# Autodesk Inventor assembly: Shooter Assembly v2
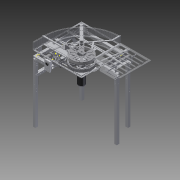
[picture p0: Inventor's stored thumbnail of the model, 180x180]
Saved by Autodesk Inventor 2013 (Build 170138000, 138)
## iProperties
Created: 2013-01-15
Part Number: Shooter Assembly v2
Document SubType Name: Assembly
Designer: actoennies
Mass: 9919.81 g
Surface Area: 30757 cm^2
Volume: 4898.75 cm^3
Density: 2.02497 g/cm^3
Author: actoennies
## Documents named in this file (53)
- C:\Users\Arpan\Documents\GitHub\frc2013CAD\Launcher\Shooter\Shooter Assembly v2.iam
- C:\Users\Arpan\Documents\GitHub\frc2013CAD\Launcher\Shooter\Bearing Mount v1.ipt
- C:\Users\Arpan\Documents\GitHub\frc2013CAD\Launcher\Shooter\Outer Rail v1.ipt
- C:\Users\Arpan\Documents\GitHub\frc2013CAD\Launcher\Shooter\Runner Rails v2.ipt
- C:\Users\Arpan\Documents\GitHub\frc2013CAD\Launcher\Shooter\Bearing.ipt
- C:\Users\Arpan\Documents\GitHub\frc2013CAD\Launcher\Shooter\Flywheel Assembly.iam
- C:\Users\Arpan\Documents\GitHub\frc2013CAD\Launcher\Shooter\Shooter Mounter.ipt
- C:\Users\Arpan\Documents\GitHub\frc2013CAD\Launcher\Shooter\Bearing Mount 2 v1.ipt
- C:\Users\Arpan\Documents\GitHub\frc2013CAD\Launcher\Shooter\Shorter Shaft.ipt
- C:\Users\Arpan\Documents\GitHub\frc2013CAD\Launcher\Shooter\Spacer Rube.ipt
- C:\Users\Arpan\Documents\GitHub\frc2013CAD\Launcher\Shooter\Edge Mount.ipt
- C:\Users\Arpan\Documents\GitHub\frc2013CAD\Launcher\Shooter\Square Tube.ipt
- C:\Users\Arpan\Documents\GitHub\frc2013CAD\Launcher\Shooter\Flange Bearing Mount Tower.ipt
- C:\Users\Arpan\Documents\GitHub\frc2013CAD\Launcher\Shooter\Flange Bearing Mount Tower Mirror.ipt
- C:\Users\Arpan\Documents\GitHub\frc2013CAD\Launcher\Shooter\Bearing Mount Top.ipt
- C:\Users\Arpan\Documents\GitHub\frc2013CAD\Launcher\Shooter\Square Motor Mount.ipt
- C:\Users\Arpan\Documents\GitHub\frc2013CAD\Launcher\Shooter\Shooter Assembly v2\Design Accelerator\Spur Gears1.iam
- C:\Users\Arpan\Documents\GitHub\frc2013CAD\Launcher\Parts\Imported Components\Snow Blower Motor\Snow Blower Motor.iam
- C:\Users\Arpan\Documents\GitHub\frc2013CAD\Launcher\Shooter\Snowblower Motor Mount.ipt
- C:\Users\Arpan\Documents\GitHub\frc2013CAD\Launcher\Shooter\8mm shaft.ipt
- C:\Users\Arpan\Documents\GitHub\frc2013CAD\Launcher\Shooter\CIM Bearing.ipt
- C:\Users\Arpan\Documents\GitHub\frc2013CAD\Launcher\Parts\8 Plaction Wheel.iam
- C:\Users\Arpan\Documents\GitHub\frc2013CAD\Launcher\Shooter\Square Tube 2.ipt
- C:\Users\Arpan\Documents\GitHub\frc2013CAD\Launcher\Parts\CIM Motor\Motors_FR801-001.iam
- C:\Users\Arpan\Documents\GitHub\frc2013CAD\Launcher\Shooter\Cim Mount.ipt
- C:\Users\Arpan\Documents\GitHub\frc2013CAD\Launcher\Shooter\Hub v1.ipt
- C:\Users\Arpan\Documents\GitHub\frc2013CAD\Launcher\Shooter\Camera Traffic Light Mount.ipt
- C:\Users\Arpan\Documents\GitHub\frc2013CAD\Launcher\Shooter\Square Tube 3.ipt
- C:\Users\Arpan\Documents\GitHub\frc2013CAD\Launcher\Shooter\edge mount shortened.ipt
- C:\Users\Arpan\Documents\GitHub\frc2013CAD\Launcher\Shooter\Camera.ipt
- C:\Users\Arpan\Documents\GitHub\frc2013CAD\Launcher\Shooter\Square Tube 6.ipt
- C:\Users\Arpan\Documents\GitHub\frc2013CAD\Launcher\Parts\NR-025_5-D(F,D-770).iam
- C:\Users\Arpan\Documents\GitHub\frc2013CAD\Launcher\Shooter\Upper Rails.ipt
- C:\Users\Arpan\Documents\GitHub\frc2013CAD\Launcher\Hopper New\Hopper Assembly.iam
- C:\Users\Arpan\Documents\GitHub\frc2013CAD\Launcher\Hopper New\Puller Mechanism.ipt
- C:\Users\Arpan\Documents\GitHub\frc2013CAD\Launcher\Shooter\Cylinder Mount 2.ipt
- C:\Users\Arpan\Documents\GitHub\frc2013CAD\Launcher\Shooter\Cylinder Mount.ipt
- C:\Users\Arpan\Documents\GitHub\frc2013CAD\Launcher\Parts\Imported Components\E3-X-315-X-D-3-X\E3-X-315-X-D-3-X.ipt
- C:\Users\Arpan\Documents\GitHub\frc2013CAD\Launcher\Shooter\Encoder Mounting.ipt
- C:\Users\Arpan\Documents\GitHub\frc2013CAD\Launcher\Hopper New\Backboard.ipt
- C:\Users\Arpan\Documents\GitHub\frc2013CAD\Launcher\Hopper New\Mount.ipt
- C:\Users\Arpan\Documents\GitHub\frc2013CAD\Launcher\Shooter\Gusset.ipt
- C:\Users\Arpan\Documents\GitHub\frc2013CAD\Launcher\Shooter\Gusset 2.ipt
- C:\Users\Arpan\Documents\GitHub\frc2013CAD\Launcher\Shooter\Gusset 3.ipt
- C:\Users\Arpan\Documents\GitHub\frc2013CAD\Launcher\Shooter\Gusset 4.ipt
- C:\Users\Arpan\Documents\GitHub\frc2013CAD\Launcher\Shooter\Inner Mount.ipt
- C:\Users\Arpan\Documents\GitHub\frc2013CAD\Launcher\Shooter\Gusset 5.ipt
- C:\Users\Arpan\Documents\GitHub\frc2013CAD\Launcher\Shooter\Hard Stop.ipt
- C:\Users\Arpan\Documents\GitHub\frc2013CAD\Launcher\Shooter\Gusset Connector 2.ipt
- C:\Users\Arpan\Documents\GitHub\frc2013CAD\Launcher\Shooter\Pneumatic Puller Mount.ipt
- C:\Users\Arpan\Documents\GitHub\frc2013CAD\Launcher\Shooter\L-Channel Strenght.ipt
- C:\Users\Arpan\Documents\GitHub\frc2013CAD\Launcher\Shooter\Gear for Angle.ipt
- C:\Users\Arpan\Documents\GitHub\frc2013CAD\Launcher\Shooter\Encoder Mount 2.ipt
## Components (78 placed, 52 different names)
1. Bearing Mount v1:1 — Insert:13, Insert:26, Insert:27, Mate:62, Mate:63, Flush:70, Insert:60, Insert:61, Mate:167
2. Outer Rail v1:1 — Insert:13, Insert:47, Insert:48, Flush:70, Mate:165
3. Runner Rails v2:1 — Insert:60, Insert:61, Mate:166, Angle:11, Flush:75, Mate:180, Mate:181, Flush:77
4. Flywheel Assembly:1 [sub-assembly] — Mate:61, Flush:30, Mate:68, Flush:31
5. Shooter Mounter:1 — Insert:26, Insert:27, Insert:34, Flush:11, Insert:35, Insert:36, Insert:37, Insert:38, Flush:19, Mate:45, Flush:40, Flush:64, Flush:72, Angle:6, Mate:176, Flush:76, Mate:183, Flush:78, Mate:226, Flush:114, Flush:115, Mate:229, Mate:230, Flush:116, Mate:232, Flush:117, Mate:236, Flush:118, Flush:119, Mate:238, Insert:75
6. Spacer Rube:1 — Insert:34, Flush:11
7. Bearing Mount 2 v1:1 — Insert:37, Insert:38, Insert:40
8. Bearing Mount 2 v1:2 — Insert:35, Insert:36, Insert:39
9. Bearing:3 — Insert:40, Flush:13, Mate:14, Mate:15
10. Bearing:4 — Insert:39, Flush:12, Mate:12, Mate:13, Mate:36, Mate:44
11. Shorter Shaft:1 — Flush:12, Mate:12, Mate:13, Mate:37
12. Shorter Shaft:2 — Flush:13, Mate:14, Mate:15, Mate:38
13. Edge Mount:2 — Flush:34, Mate:104, Flush:48, Mate:106, Flush:68, Mate:174, Flush:74, Mate:220, Mate:222
14. Square Tube:2 — Flush:19, Flush:23, Mate:52, Flush:27, Mate:81, Flush:32, Mate:93, Flush:41, Flush:42, Mate:125, Mate:126, Mate:130, Flush:50, Mate:169, Mate:192, Flush:83, Mate:203, Flush:88, Mate:214, Mate:217, Flush:103, Flush:112, Insert:71, Insert:72
15. Flange Bearing Mount Tower:1 — Insert:43, Flush:112, Flush:113
16. Bearing:5 — Insert:43, Mate:36, Mate:37
17. Flange Bearing Mount Tower Mirror:1 — Flush:55, Mate:135, Flush:111, Insert:70
18. Bearing:6 — Mate:38, Insert:70
19. Bearing Mount Top:1 — Insert:47, Insert:48, Mate:65, Mate:66, Mate:68, Mate:162, Mate:163, Mate:164
20. Square Motor Mount:1 — Flush:23, Mate:47, Mate:51, Flush:27, Mate:131, Mate:197, Mate:198, Flush:86, Flush:96, Flush:106
21. Spur Gears:1 [sub-assembly] — Mate:44, Mate:45, Flush:25, Mate:46, Angle:2, Flush:64, Angle:6, Angle:10, Mate:227, Mate:228, Mate:231, Mate:233, Flush:120, Mate:239
22. Snow Blower Motor:1 [sub-assembly] — Flush:25, Mate:46, Angle:2, Insert:50, Insert:51
23. Snowblower Motor Mount:1 — Insert:50, Insert:51, Mate:47, Mate:51, Mate:52, Mate:240, Insert:76, Insert:78, Insert:79
24. 8mm shaft:1 — Mate:61, Flush:30, Mate:67, Flush:31, Mate:82, Mate:83, Mate:84, Mate:86, Mate:167, Insert:64
25. CIM Bearing:1 — Mate:65, Mate:66, Mate:67
26. CIM Bearing:2 — Mate:62, Mate:63, Insert:56
27. 8 Plaction Wheel:1 [sub-assembly] — Mate:88, Mate:89, Mate:90, Mate:91, Mate:92
28. Square Tube 2:1 — Mate:81, Flush:32, Flush:34, Mate:106, Mate:124, Flush:49, Mate:126, Mate:173, Mate:186, Flush:80, Mate:193, Mate:216, Mate:219, Flush:104, Flush:111, Flush:113
29. Motors_FR801-001:1 [sub-assembly] — Mate:82, Mate:83, Mate:84, Mate:143, Mate:144, Mate:145
30. Cim Mount:1 — Flush:40, Mate:143, Mate:144, Mate:145
31. Hub v1:1 — Mate:88, Mate:89, Mate:90, Flush:38
32. Hub v1:2 — Mate:91, Flush:38, Mate:92, Insert:56
33. Camera Traffic Light Mount:1 — Mate:93, Flush:41, Flush:42, Mate:127, Mate:128, Mate:129, Mate:202, Mate:211, Angle:15
34. Square Tube 3:1 — Mate:104, Flush:48, Flush:55, Mate:135, Mate:173, Mate:174, Flush:74, Mate:175, Mate:187, Mate:206, Flush:90, Mate:221, Flush:105, Flush:110
35. edge mount shortened:1 — Mate:124, Mate:125, Flush:49, Mate:196, Flush:85, Mate:215, Flush:102, Mate:218, Mate:223, Flush:107
36. Camera:1 — Mate:127, Mate:128, Mate:129
37. Edge Mount:3 — Mate:130, Mate:131, Flush:50, Mate:199, Mate:209, Flush:97, Mate:212, Flush:100, Mate:213, Flush:101
38. Square Tube 6:1 — Mate:175, Flush:91, Mate:207, Flush:93, Mate:208, Flush:94, Flush:95, Flush:110, Mate:224, Insert:73, Insert:74
39. Upper Rails:1 — Mate:162, Mate:163, Mate:164
40. Hopper Assembly:1 [sub-assembly] — Flush:72, Mate:165, Mate:166, Flush:75, Angle:12, Mate:178, Mate:179
41. Puller Mechanism:1 — Insert:69, Angle:12, Mate:237
42. Cylinder Mount 2:1 — Angle:10, Mate:169, Angle:13, Mate:182, Mate:183, Flush:78
43. Cylinder Mount:1 — Mate:176, Flush:76, Mate:177, Insert:66, Insert:67
44. E3-X-315-X-D-3-X:1 — Insert:64, Insert:65
45. Encoder Mounting:1 — Insert:65, Angle:11
46. NR-025_5-D(F,D-770):1 [sub-assembly] — Mate:177, Insert:66, Insert:67, Insert:69, Angle:13, Mate:182
47. Backboard:1 — Mate:178, Mate:179
48. Mount:1 — Mate:180, Mate:181, Flush:77
49. Gusset:3 — Mate:186, Flush:80, Mate:187
50. Gusset:4 — Mate:196, Mate:197, Flush:85
51. Gusset:5 — Mate:192, Mate:193, Flush:83
52. Gusset:8 — Mate:198, Mate:199, Flush:86
53. Gusset:10 — Mate:202, Mate:203, Flush:88
54. Gusset 2:1 — Mate:206, Flush:90, Flush:91
55. Gusset 3:2 — Mate:209, Flush:96, Flush:97
56. Gusset 3:3 — Mate:208, Flush:94, Flush:95, Flush:108
57. Gusset 3:4 — Mate:207, Flush:93, Mate:225
58. Gusset 4:1 — Mate:211, Mate:212, Flush:100
59. Gusset 4:2 — Mate:213, Flush:101, Mate:214
60. Gusset 4:3 — Mate:217, Mate:218, Flush:103
61. Gusset 4:4 — Mate:215, Flush:102, Mate:216
62. Gusset 4:5 — Mate:219, Mate:220, Flush:104
63. Gusset 4:6 — Mate:221, Mate:222, Flush:105
64. Gusset 3:5 — Mate:223, Flush:106, Flush:107
65. Inner Mount:1 — Flush:108, Mate:224, Mate:225
66. Gusset 5:1 — Flush:115, Mate:228, Mate:229
67. Gusset 5:2 — Mate:226, Mate:227, Flush:114
68. Gusset 5:3 — Mate:230, Mate:231, Flush:116
69. Gusset 5:4 — Mate:232, Mate:233, Flush:117
70. Hard Stop:1 — Insert:71, Insert:72
71. Gusset Connector 2:1 — Insert:73, Insert:74
72. Pneumatic Puller Mount:1 — Mate:236, Flush:118, Mate:237
73. L-Channel Strenght:1 — Flush:119, Mate:238, Insert:75, Angle:15
74. Gear for Angle:1 — Flush:120, Mate:239, Mate:240, Flush:121
75. CIM Bearing:3 — Insert:76, Insert:77
76. 8mm shaft:2 — Insert:77, Flush:121
77. E3-X-315-X-D-3-X:2 — Insert:80, Angle:14
78. Encoder Mount 2:1 — Insert:78, Insert:79, Insert:80, Angle:14
## Relationships (208: Mate 105, Flush 61, Insert 34, Angle 8)
- Insert:13: Bearing Mount v1:1 ↔ Outer Rail v1:1
- Insert:26: Bearing Mount v1:1 ↔ Shooter Mounter:1
- Insert:27: Bearing Mount v1:1 ↔ Shooter Mounter:1
- Insert:34: Shooter Mounter:1 ↔ Spacer Rube:1
- Flush:11: Shooter Mounter:1 ↔ Spacer Rube:1
- Insert:35: Shooter Mounter:1 ↔ Bearing Mount 2 v1:2
- Insert:36: Shooter Mounter:1 ↔ Bearing Mount 2 v1:2
- Insert:37: Shooter Mounter:1 ↔ Bearing Mount 2 v1:1
- Insert:38: Shooter Mounter:1 ↔ Bearing Mount 2 v1:1
- Insert:39: Bearing Mount 2 v1:2 ↔ Bearing:4
- Insert:40: Bearing Mount 2 v1:1 ↔ Bearing:3
- Flush:12 (-25.4 mm): Bearing:4 ↔ Shorter Shaft:1
- Mate:12: Bearing:4 ↔ Shorter Shaft:1
- Mate:13: Bearing:4 ↔ Shorter Shaft:1
- Flush:13 (-25.4 mm): Bearing:3 ↔ Shorter Shaft:2
- Mate:14: Bearing:3 ↔ Shorter Shaft:2
- Mate:15: Bearing:3 ↔ Shorter Shaft:2
- Insert:43: Flange Bearing Mount Tower:1 ↔ Bearing:5
- Flush:19: Shooter Mounter:1 ↔ Square Tube:2
- Mate:36: Bearing:4 ↔ Bearing:5
- Mate:37: Shorter Shaft:1 ↔ Bearing:5
- Mate:38: Shorter Shaft:2 ↔ Bearing:6
- Insert:47: Outer Rail v1:1 ↔ Bearing Mount Top:1
- Insert:48: Outer Rail v1:1 ↔ Bearing Mount Top:1
- Flush:23 (152.4 mm): Square Tube:2 ↔ Square Motor Mount:1
- Mate:44: Bearing:4 ↔ Spur Gears:1
- Mate:45 (25.4 mm): Shooter Mounter:1 ↔ Spur Gears:1
- Flush:25 (-3.175 mm): Spur Gears:1 ↔ Snow Blower Motor:1
- Mate:46: Spur Gears:1 ↔ Snow Blower Motor:1
- Angle:2 (0 deg): Spur Gears:1 ↔ Snow Blower Motor:1
- Insert:50: Snow Blower Motor:1 ↔ Snowblower Motor Mount:1
- Insert:51: Snow Blower Motor:1 ↔ Snowblower Motor Mount:1
- Mate:47: Square Motor Mount:1 ↔ Snowblower Motor Mount:1
- Mate:51: Square Motor Mount:1 ↔ Snowblower Motor Mount:1
- Mate:52: Square Tube:2 ↔ Snowblower Motor Mount:1
- Flush:27: Square Tube:2 ↔ Square Motor Mount:1
- Mate:61: Flywheel Assembly:1 ↔ 8mm shaft:1
- Flush:30 (12.7 mm): Flywheel Assembly:1 ↔ 8mm shaft:1
- Mate:62: Bearing Mount v1:1 ↔ CIM Bearing:2
- Mate:63: Bearing Mount v1:1 ↔ CIM Bearing:2
- Mate:65: Bearing Mount Top:1 ↔ CIM Bearing:1
- Mate:66: Bearing Mount Top:1 ↔ CIM Bearing:1
- Mate:67: 8mm shaft:1 ↔ CIM Bearing:1
- Mate:68 (6.35 mm): Flywheel Assembly:1 ↔ Bearing Mount Top:1
- Flush:31: Flywheel Assembly:1 ↔ 8mm shaft:1
- Mate:81: Square Tube:2 ↔ Square Tube 2:1
- Flush:32: Square Tube:2 ↔ Square Tube 2:1
- Flush:34: Edge Mount:2 ↔ Square Tube 2:1
- Mate:82: 8mm shaft:1 ↔ Motors_FR801-001:1
- Mate:83: 8mm shaft:1 ↔ Motors_FR801-001:1
- Mate:84: 8mm shaft:1 ↔ Motors_FR801-001:1
- Mate:86: 8mm shaft:1
- Mate:88: 8 Plaction Wheel:1 ↔ Hub v1:1
- Mate:89: 8 Plaction Wheel:1 ↔ Hub v1:1
- Mate:90: 8 Plaction Wheel:1 ↔ Hub v1:1
- Mate:91: 8 Plaction Wheel:1 ↔ Hub v1:2
- Flush:38: Hub v1:1 ↔ Hub v1:2
- Mate:92: 8 Plaction Wheel:1 ↔ Hub v1:2
- Insert:56: CIM Bearing:2 ↔ Hub v1:2
- Flush:40: Shooter Mounter:1 ↔ Cim Mount:1
- Mate:93: Square Tube:2 ↔ Camera Traffic Light Mount:1
- Flush:41: Square Tube:2 ↔ Camera Traffic Light Mount:1
- Flush:42: Square Tube:2 ↔ Camera Traffic Light Mount:1
- Mate:104: Edge Mount:2 ↔ Square Tube 3:1
- Flush:48: Edge Mount:2 ↔ Square Tube 3:1
- Mate:106: Edge Mount:2 ↔ Square Tube 2:1
- Mate:124: Square Tube 2:1 ↔ edge mount shortened:1
- Mate:125: Square Tube:2 ↔ edge mount shortened:1
- Flush:49: Square Tube 2:1 ↔ edge mount shortened:1
- Mate:126: Square Tube:2 ↔ Square Tube 2:1
- Mate:127: Camera Traffic Light Mount:1 ↔ Camera:1
- Mate:128: Camera Traffic Light Mount:1 ↔ Camera:1
- Mate:129: Camera Traffic Light Mount:1 ↔ Camera:1
- Mate:130: Square Tube:2 ↔ Edge Mount:3
- Mate:131: Square Motor Mount:1 ↔ Edge Mount:3
- Flush:50: Square Tube:2 ↔ Edge Mount:3
- Flush:55: Flange Bearing Mount Tower Mirror:1 ↔ Square Tube 3:1
- Mate:135: Flange Bearing Mount Tower Mirror:1 ↔ Square Tube 3:1
- Mate:143: Motors_FR801-001:1 ↔ Cim Mount:1
- Mate:144: Motors_FR801-001:1 ↔ Cim Mount:1
- Mate:145: Motors_FR801-001:1 ↔ Cim Mount:1
- Flush:64 (3.175 mm): Shooter Mounter:1 ↔ Spur Gears:1
- Mate:162: Bearing Mount Top:1 ↔ Upper Rails:1
- Mate:163: Bearing Mount Top:1 ↔ Upper Rails:1
- Mate:164: Bearing Mount Top:1 ↔ Upper Rails:1
- Flush:68 (-950.9125 mm): Edge Mount:2
- Flush:70: Bearing Mount v1:1 ↔ Outer Rail v1:1
- Flush:72: Shooter Mounter:1 ↔ Hopper Assembly:1
- Insert:60: Bearing Mount v1:1 ↔ Runner Rails v2:1
- Insert:61: Bearing Mount v1:1 ↔ Runner Rails v2:1
- Mate:165: Outer Rail v1:1 ↔ Hopper Assembly:1
- Mate:166: Runner Rails v2:1 ↔ Hopper Assembly:1
- Angle:6 (180 deg): Shooter Mounter:1 ↔ Spur Gears:1
- Mate:167: Bearing Mount v1:1 ↔ 8mm shaft:1
- Angle:10 (0 deg): Spur Gears:1 ↔ Cylinder Mount 2:1
- Mate:169 (101.6 mm): Square Tube:2 ↔ Cylinder Mount 2:1
- Insert:64 (3.175 mm): 8mm shaft:1 ↔ E3-X-315-X-D-3-X:1
- Mate:173: Square Tube 2:1 ↔ Square Tube 3:1
- Mate:174: Edge Mount:2 ↔ Square Tube 3:1
- Flush:74: Edge Mount:2 ↔ Square Tube 3:1
- Mate:175: Square Tube 3:1 ↔ Square Tube 6:1
- Insert:65: E3-X-315-X-D-3-X:1 ↔ Encoder Mounting:1
- Angle:11 (180 deg): Runner Rails v2:1 ↔ Encoder Mounting:1
- Flush:75: Runner Rails v2:1 ↔ Hopper Assembly:1
- Mate:176: Shooter Mounter:1 ↔ Cylinder Mount:1
- Flush:76: Shooter Mounter:1 ↔ Cylinder Mount:1
- Mate:177: Cylinder Mount:1 ↔ NR-025_5-D(F,D-770):1
- Insert:66: Cylinder Mount:1 ↔ NR-025_5-D(F,D-770):1
- Insert:67: Cylinder Mount:1 ↔ NR-025_5-D(F,D-770):1
- Insert:69 (3.175 mm): Puller Mechanism:1 ↔ NR-025_5-D(F,D-770):1
- Angle:12 (0 deg): Hopper Assembly:1 ↔ Puller Mechanism:1
- Mate:178: Hopper Assembly:1 ↔ Backboard:1
- Mate:179: Hopper Assembly:1 ↔ Backboard:1
- Mate:180: Runner Rails v2:1 ↔ Mount:1
- Mate:181: Runner Rails v2:1 ↔ Mount:1
- Flush:77: Runner Rails v2:1 ↔ Mount:1
- Angle:13 (0 deg): Cylinder Mount 2:1 ↔ NR-025_5-D(F,D-770):1
- Mate:182: Cylinder Mount 2:1 ↔ NR-025_5-D(F,D-770):1
- Mate:183: Shooter Mounter:1 ↔ Cylinder Mount 2:1
- Flush:78: Shooter Mounter:1 ↔ Cylinder Mount 2:1
- Mate:186: Square Tube 2:1 ↔ Gusset:3
- Flush:80: Square Tube 2:1 ↔ Gusset:3
- Mate:187: Square Tube 3:1 ↔ Gusset:3
- Mate:192: Square Tube:2 ↔ Gusset:5
- Mate:193: Square Tube 2:1 ↔ Gusset:5
- Flush:83: Square Tube:2 ↔ Gusset:5
- Mate:196: edge mount shortened:1 ↔ Gusset:4
- Mate:197: Square Motor Mount:1 ↔ Gusset:4
- Flush:85: edge mount shortened:1 ↔ Gusset:4
- Mate:198: Square Motor Mount:1 ↔ Gusset:8
- Mate:199: Edge Mount:3 ↔ Gusset:8
- Flush:86: Square Motor Mount:1 ↔ Gusset:8
- Mate:202: Camera Traffic Light Mount:1 ↔ Gusset:10
- Mate:203: Square Tube:2 ↔ Gusset:10
- Flush:88: Square Tube:2 ↔ Gusset:10
- Mate:206: Square Tube 3:1 ↔ Gusset 2:1
- Flush:90: Square Tube 3:1 ↔ Gusset 2:1
- Flush:91: Square Tube 6:1 ↔ Gusset 2:1
- Mate:207: Square Tube 6:1 ↔ Gusset 3:4
- Flush:93: Square Tube 6:1 ↔ Gusset 3:4
- Mate:208: Square Tube 6:1 ↔ Gusset 3:3
- Flush:94: Square Tube 6:1 ↔ Gusset 3:3
- Flush:95: Square Tube 6:1 ↔ Gusset 3:3
- Mate:209: Edge Mount:3 ↔ Gusset 3:2
- Flush:96: Square Motor Mount:1 ↔ Gusset 3:2
- Flush:97: Edge Mount:3 ↔ Gusset 3:2
- Mate:211: Camera Traffic Light Mount:1 ↔ Gusset 4:1
- Mate:212: Edge Mount:3 ↔ Gusset 4:1
- Flush:100: Edge Mount:3 ↔ Gusset 4:1
- Mate:213: Edge Mount:3 ↔ Gusset 4:2
- Flush:101: Edge Mount:3 ↔ Gusset 4:2
- Mate:214: Square Tube:2 ↔ Gusset 4:2
- Mate:215: edge mount shortened:1 ↔ Gusset 4:4
- Flush:102: edge mount shortened:1 ↔ Gusset 4:4
- Mate:216: Square Tube 2:1 ↔ Gusset 4:4
- Mate:217: Square Tube:2 ↔ Gusset 4:3
- Mate:218: edge mount shortened:1 ↔ Gusset 4:3
- Flush:103: Square Tube:2 ↔ Gusset 4:3
- Mate:219: Square Tube 2:1 ↔ Gusset 4:5
- Mate:220: Edge Mount:2 ↔ Gusset 4:5
- Flush:104: Square Tube 2:1 ↔ Gusset 4:5
- Mate:221: Square Tube 3:1 ↔ Gusset 4:6
- Mate:222: Edge Mount:2 ↔ Gusset 4:6
- Flush:105: Square Tube 3:1 ↔ Gusset 4:6
- Mate:223: edge mount shortened:1 ↔ Gusset 3:5
- Flush:106: Square Motor Mount:1 ↔ Gusset 3:5
- Flush:107: edge mount shortened:1 ↔ Gusset 3:5
- Flush:108: Gusset 3:3 ↔ Inner Mount:1
- Flush:110: Square Tube 3:1 ↔ Square Tube 6:1
- Mate:224: Square Tube 6:1 ↔ Inner Mount:1
- Mate:225: Gusset 3:4 ↔ Inner Mount:1
- Flush:111: Flange Bearing Mount Tower Mirror:1 ↔ Square Tube 2:1
- Flush:112: Square Tube:2 ↔ Flange Bearing Mount Tower:1
- Flush:113: Flange Bearing Mount Tower:1 ↔ Square Tube 2:1
- Insert:70: Flange Bearing Mount Tower Mirror:1 ↔ Bearing:6
- Mate:226: Shooter Mounter:1 ↔ Gusset 5:2
- Mate:227: Spur Gears:1 ↔ Gusset 5:2
- Flush:114: Shooter Mounter:1 ↔ Gusset 5:2
- Flush:115: Shooter Mounter:1 ↔ Gusset 5:1
- Mate:228: Spur Gears:1 ↔ Gusset 5:1
- Mate:229: Shooter Mounter:1 ↔ Gusset 5:1
- Mate:230: Shooter Mounter:1 ↔ Gusset 5:3
- Mate:231: Spur Gears:1 ↔ Gusset 5:3
- Flush:116: Shooter Mounter:1 ↔ Gusset 5:3
- Mate:232: Shooter Mounter:1 ↔ Gusset 5:4
- Mate:233: Spur Gears:1 ↔ Gusset 5:4
- Flush:117: Shooter Mounter:1 ↔ Gusset 5:4
- Insert:71: Square Tube:2 ↔ Hard Stop:1
- Insert:72: Square Tube:2 ↔ Hard Stop:1
- Insert:73: Square Tube 6:1 ↔ Gusset Connector 2:1
- Insert:74: Square Tube 6:1 ↔ Gusset Connector 2:1
- Mate:236: Shooter Mounter:1 ↔ Pneumatic Puller Mount:1
- Flush:118: Shooter Mounter:1 ↔ Pneumatic Puller Mount:1
- Mate:237 (18.415 mm): Puller Mechanism:1 ↔ Pneumatic Puller Mount:1
- Flush:119: Shooter Mounter:1 ↔ L-Channel Strenght:1
- Mate:238: Shooter Mounter:1 ↔ L-Channel Strenght:1
- Insert:75: Shooter Mounter:1 ↔ L-Channel Strenght:1
- Flush:120: Spur Gears:1 ↔ Gear for Angle:1
- Mate:239 (304.8 mm): Spur Gears:1 ↔ Gear for Angle:1
- Mate:240: Snowblower Motor Mount:1 ↔ Gear for Angle:1
- Insert:76: Snowblower Motor Mount:1 ↔ CIM Bearing:3
- Insert:77 (-3.175 mm): CIM Bearing:3 ↔ 8mm shaft:2
- Flush:121: Gear for Angle:1 ↔ 8mm shaft:2
- Insert:78: Snowblower Motor Mount:1 ↔ Encoder Mount 2:1
- Insert:79: Snowblower Motor Mount:1 ↔ Encoder Mount 2:1
- Insert:80: E3-X-315-X-D-3-X:2 ↔ Encoder Mount 2:1
- Angle:14 (180 deg): E3-X-315-X-D-3-X:2 ↔ Encoder Mount 2:1
- Angle:15 (180 deg): Camera Traffic Light Mount:1 ↔ L-Channel Strenght:1
